# Autodesk Inventor assembly: boardC
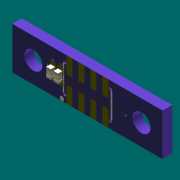
[picture p0: Inventor's stored thumbnail of the model, 180x180]
Saved by Autodesk Inventor 2016 (Build 200138000, 138)
## iProperties
Created: 2016-02-15
Part Number: boardC
Document SubType Name: Assembly
Designer: sawai
Author: sawai
## Documents named in this file (4)
- C:\Users\Jonathan\Documents\Projects\mppcSensor\cad\sensorBoardC\boardC.iam
- C:\Users\Jonathan\Documents\Projects\mppcSensor\cad\sensorBoardC\pcb.ipt
- C:\Users\Jonathan\Documents\Projects\mppcSensor\cad\electronics\capacitor-0603.ipt
- C:\Users\sawaiz\OneDrive\projects\mppcSensor\cad\electronics\capacitor.ipt
## Components (3 placed, 2 different names)
1. pcb:1 — Mate:1
2. capacitor-0603:1 — Flush:1, Flush:2
3. capacitor-0603:2 — Flush:1, Flush:2, Mate:1
## Relationships (3: Flush 2, Mate 1)
- Flush:1: capacitor-0603:1 ↔ capacitor-0603:2
- Flush:2: capacitor-0603:1 ↔ capacitor-0603:2
- Mate:1: pcb:1 ↔ capacitor-0603:2
